# Autodesk Inventor assembly: pinballAssembly
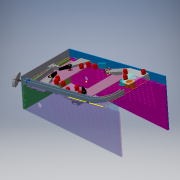
[picture p0: Inventor's stored thumbnail of the model, 180x180]
Saved by Autodesk Inventor 2017 (Build 210142000, 142)
## iProperties
Created: 2017-02-19
Part Number: pinballAssembly
Document SubType Name: Assembly
Designer: John
Author: John
## Documents named in this file (34)
- C:\Users\John\Dropbox\ECE115\pinball-project\pinballAssembly.iam
- C:\Users\John\Dropbox\ECE115\pinball-project\playfield.ipt
- C:\Users\John\Dropbox\ECE115\pinball-project\modular-post.ipt
- C:\Users\John\Dropbox\ECE115\module-2\paddle2.ipt
- C:\Users\John\Dropbox\ECE115\pinball-project\part_pinball_ece115.ipt
- C:\Users\John\Dropbox\ECE115\pinball-project\flipper-hug-left.ipt
- C:\Users\John\Dropbox\ECE115\pinball-project\thumper-bumper-assm-v3.iam
- C:\Users\John\Dropbox\ECE115\pinball-project\pinball-case-left-wall.ipt
- C:\Users\John\Dropbox\ECE115\pinball-project\pinball-case-left-wall-outer.ipt
- C:\Users\John\Dropbox\ECE115\pinball-project\wall-front.ipt
- C:\Users\John\Dropbox\ECE115\pinball-project\wall-front-outer.ipt
- C:\Users\John\Dropbox\ECE115\pinball-project\plunger-curve-outer.ipt
- C:\Users\John\Dropbox\ECE115\pinball-project\plunger-curve-inner.ipt
- C:\Users\John\Dropbox\ECE115\pinball-project\ball-reload-right.ipt
- C:\Users\John\Dropbox\ECE115\pinball-project\ball-waterfall.ipt
- C:\Users\John\Dropbox\ECE115\pinball-project\ramp-support.ipt
- C:\Users\John\Dropbox\ECE115\pinball-project\flipper-support.ipt
- C:\Users\John\Dropbox\ECE115\module-2\rod.ipt
- C:\Users\John\Dropbox\ECE115\module-2\Solenoid 1240S\Solenoid.iam
- C:\Users\John\Dropbox\ECE115\pinball-project\pinball-case-back.ipt
- C:\Users\John\Dropbox\ECE115\pinball-project\game-over.ipt
- C:\Users\John\Dropbox\ECE115\pinball-project\flipper-hug-left-2.ipt
- C:\Users\John\Downloads\level2.ipt
- C:\Users\John\Downloads\funil.ipt
- C:\Users\John\Downloads\ramp.ipt
- C:\Users\John\Downloads\ServoMotor.ipt
- C:\Users\John\Downloads\GATE servo motor.ipt
- C:\Users\John\Downloads\wall-outer-plunger-updated.ipt
- C:\Users\John\Downloads\wall-inner-plunger-updated.ipt
- C:\Users\John\Downloads\plunger-support.ipt
- C:\Users\John\Downloads\Handle_plunger.ipt
- C:\Users\John\Dropbox\ECE115\pinball-project\flipper-support2.ipt
- C:\Users\John\Dropbox\ECE115\module-2\flipper-bottom.ipt
- C:\Users\John\Dropbox\ECE115\module-2\interstitial-flipper.ipt
## Components (59 placed, 33 different names)
1. playfield:1 — Mate:1, Mate:2, Tangent:1, Mate:10, Insert:4, Insert:5, Insert:6, Flush:8, Mate:16, Flush:18, Tangent:3, Mate:29, Mate:30, Mate:31, Mate:34, Mate:41, Angle:8, Mate:42, Mate:50, Mate:51, Mate:54, Mate:55, Angle:12, Angle:13, Angle:14, Mate:65, Mate:66, Flush:34, Mate:67, Mate:68, Mate:69, Mate:76, Angle:17, Flush:35, Mate:80, Angle:18, Mate:83, Mate:85, Mate:86, Mate:87, Flush:36, Mate:88, Mate:89, Mate:90, Mate:96, Rotational:11, Mate:121, Mate:122, Mate:123
2. modular-post:1 — Insert:5
3. modular-post:2 — Insert:4
4. modular-post:3 — Insert:6
5. paddle2:1 — Mate:1, Mate:55, Mate:56, Mate:77
6. paddle2:2 — Mate:2, Rotational:4, Mate:54, Mate:57, Flush:31
7. part_pinball_ece115:1 — Tangent:1
8. flipper-hug-left:2 — Mate:10, Rotational:4, Angle:12
9. modular-post:4
10. modular-post:5
11. modular-post:6
12. thumper-bumper-assm-v3:1 [sub-assembly] — Mate:65, Mate:66, Flush:34
13. thumper-bumper-assm-v3:2 [sub-assembly] — Flush:8, Mate:67, Mate:68
14. pinball-case-left-wall:1 — Mate:16, Flush:23, Flush:24, Flush:25, Mate:47, Flush:29, Mate:49, Mate:50, Mate:51, Flush:30, Mate:52, Mate:53, Angle:19, Mate:102, Mate:104, Mate:105
15. pinball-case-left-wall-outer:1 — Flush:25, Mate:47, Flush:26, Flush:27, Angle:15, Mate:79, Mate:82
16. wall-front:1 — Flush:15, Flush:17, Mate:22, Flush:23, Flush:24, Flush:28, Mate:48, Mate:49, Angle:21
17. pinball-case-left-wall-outer:2 — Flush:15, Tangent:2, Angle:4, Tangent:4, Flush:27, Mate:75
18. wall-front-outer:1 — Flush:17, Flush:18, Mate:22, Flush:26
19. plunger-curve-outer:1 — Tangent:2, Angle:4, Tangent:3, Angle:5, Flush:22
20. plunger-curve-inner:1 — Angle:5, Tangent:4, Flush:22
21. modular-post:7 — Mate:29
22. modular-post:8 — Mate:30
23. modular-post:10 — Mate:31
24. paddle2:3 — Mate:34, Mate:101, Flush:38, Rotational:11
25. ball-reload-right:1 — Mate:121, Mate:122, Mate:123
26. ball-waterfall:1 — Mate:41, Angle:8, Mate:78
27. ramp-support:1 — Mate:42, Flush:39, Mate:106
28. pinball-case-left-wall:2 — Flush:28, Flush:29, Mate:48, Flush:32, Mate:61, Mate:62, Mate:75
29. flipper-support:1 — Flush:30, Mate:52, Mate:53, Mate:59, Mate:109, Mate:110
30. rod:1 — Mate:57, Flush:31, Mate:112
31. rod:2 — Mate:56, Mate:115
32. Solenoid:1 [sub-assembly] — Mate:59, Angle:13, Mate:109, Rotational:13
33. pinball-case-back:1 — Angle:14, Flush:32, Mate:61, Mate:62
34. game-over:1 — Mate:69, Angle:15
35. flipper-hug-left-2:1 — Mate:76, Angle:17, Mate:77
36. level2:1 — Mate:78, Mate:79, Flush:35, Mate:81, Rotational:7, Rotational:8, Rotational:9, Mate:84
37. funil:1 — Mate:80, Mate:81, Angle:18
38. modular-post:12 — Rotational:7
39. modular-post:13 — Rotational:8
40. modular-post:14 — Rotational:9
41. ramp:1 — Mate:82, Mate:83, Mate:84, Flush:39, Mate:106
42. ServoMotor:1 — Mate:85, Angle:19, Mate:86, Rotational:10
43. GATE servo motor:1 — Rotational:10
44. wall-outer-plunger-updated:1 — Mate:87, Flush:36, Mate:88, Mate:91, Mate:93, Mate:94, Flush:37
45. wall-inner-plunger-updated:1 — Mate:89, Mate:90, Mate:91
46. plunger-support:1 — Mate:93, Mate:94, Flush:37, Mate:95, Angle:20
47. Handle_plunger:1 — Mate:95, Angle:20, Mate:96, Mate:97, Mate:98
48. rod:3 — Mate:97, Mate:98, Mate:99, Mate:100
49. rod:4 — Mate:99, Mate:100
50. rod:5 — Mate:101, Flush:38, Mate:118
51. flipper-support2:1 — Mate:102, Mate:104, Mate:105, Mate:111
52. Solenoid:2 [sub-assembly] — Mate:110, Angle:21, Rotational:12
53. Solenoid:3 [sub-assembly] — Mate:111, Rotational:14
54. flipper-bottom:1 — Mate:115, Mate:116, Mate:117
55. flipper-bottom:2 — Mate:112, Mate:113, Mate:114
56. flipper-bottom:3 — Mate:118, Mate:119, Mate:120
57. interstitial-flipper:1 — Rotational:12, Mate:113, Mate:114
58. interstitial-flipper:2 — Rotational:14, Mate:119, Mate:120
59. interstitial-flipper:3 — Rotational:13, Mate:116, Mate:117
## Relationships (124: Mate 75, Flush 21, Angle 12, RevoluteJoint 9, Tangent 4, Insert 3)
- Mate:1: playfield:1 ↔ paddle2:1
- Mate:2: playfield:1 ↔ paddle2:2
- Tangent:1: playfield:1 ↔ part_pinball_ece115:1
- Mate:10: playfield:1 ↔ flipper-hug-left:2
- Rotational:4 [RevoluteJoint]: paddle2:2 ↔ flipper-hug-left:2
- Insert:4: playfield:1 ↔ modular-post:2
- Insert:5: playfield:1 ↔ modular-post:1
- Insert:6: playfield:1 ↔ modular-post:3
- Flush:8: playfield:1 ↔ thumper-bumper-assm-v3:2
- Mate:16: playfield:1 ↔ pinball-case-left-wall:1
- Flush:15: wall-front:1 ↔ pinball-case-left-wall-outer:2
- Flush:17: wall-front:1 ↔ wall-front-outer:1
- Flush:18 (-3 mm): playfield:1 ↔ wall-front-outer:1
- Mate:22: wall-front:1 ↔ wall-front-outer:1
- Tangent:2: pinball-case-left-wall-outer:2 ↔ plunger-curve-outer:1
- Angle:4 (90 deg): pinball-case-left-wall-outer:2 ↔ plunger-curve-outer:1
- Tangent:3: playfield:1 ↔ plunger-curve-outer:1
- Angle:5 (0 deg): plunger-curve-outer:1 ↔ plunger-curve-inner:1
- Tangent:4 (20 mm): pinball-case-left-wall-outer:2 ↔ plunger-curve-inner:1
- Flush:22: plunger-curve-outer:1 ↔ plunger-curve-inner:1
- Mate:29: playfield:1 ↔ modular-post:7
- Mate:30: playfield:1 ↔ modular-post:8
- Mate:31: playfield:1 ↔ modular-post:10
- Mate:34: playfield:1 ↔ paddle2:3
- Mate:41: playfield:1 ↔ ball-waterfall:1
- Angle:8 (15 deg): playfield:1 ↔ ball-waterfall:1
- Mate:42: playfield:1 ↔ ramp-support:1
- Flush:23: pinball-case-left-wall:1 ↔ wall-front:1
- Flush:24: pinball-case-left-wall:1 ↔ wall-front:1
- Flush:25: pinball-case-left-wall:1 ↔ pinball-case-left-wall-outer:1
- Mate:47: pinball-case-left-wall:1 ↔ pinball-case-left-wall-outer:1
- Flush:26 (3 mm): pinball-case-left-wall-outer:1 ↔ wall-front-outer:1
- Flush:27: pinball-case-left-wall-outer:1 ↔ pinball-case-left-wall-outer:2
- Flush:28: wall-front:1 ↔ pinball-case-left-wall:2
- Flush:29: pinball-case-left-wall:1 ↔ pinball-case-left-wall:2
- Mate:48: wall-front:1 ↔ pinball-case-left-wall:2
- Mate:49: pinball-case-left-wall:1 ↔ wall-front:1
- Mate:50: playfield:1 ↔ pinball-case-left-wall:1
- Mate:51: playfield:1 ↔ pinball-case-left-wall:1
- Flush:30: pinball-case-left-wall:1 ↔ flipper-support:1
- Mate:52: pinball-case-left-wall:1 ↔ flipper-support:1
- Mate:53: pinball-case-left-wall:1 ↔ flipper-support:1
- Mate:54: playfield:1 ↔ paddle2:2
- Mate:55: playfield:1 ↔ paddle2:1
- Angle:12 (0 deg): playfield:1 ↔ flipper-hug-left:2
- Mate:56: paddle2:1 ↔ rod:2
- Mate:57: paddle2:2 ↔ rod:1
- Flush:31: paddle2:2 ↔ rod:1
- Mate:59: flipper-support:1 ↔ Solenoid:1
- Angle:13 (180 deg): playfield:1 ↔ Solenoid:1
- Angle:14 (0 deg): playfield:1 ↔ pinball-case-back:1
- Flush:32: pinball-case-left-wall:2 ↔ pinball-case-back:1
- Mate:61: pinball-case-left-wall:2 ↔ pinball-case-back:1
- Mate:62: pinball-case-left-wall:2 ↔ pinball-case-back:1
- Mate:65: playfield:1 ↔ thumper-bumper-assm-v3:1
- Mate:66: playfield:1 ↔ thumper-bumper-assm-v3:1
- Flush:34: playfield:1 ↔ thumper-bumper-assm-v3:1
- Mate:67: playfield:1 ↔ thumper-bumper-assm-v3:2
- Mate:68: playfield:1 ↔ thumper-bumper-assm-v3:2
- Mate:69: playfield:1 ↔ game-over:1
- Angle:15 (180 deg): pinball-case-left-wall-outer:1 ↔ game-over:1
- Mate:75: pinball-case-left-wall-outer:2 ↔ pinball-case-left-wall:2
- Mate:76: playfield:1 ↔ flipper-hug-left-2:1
- Angle:17 (0 deg): playfield:1 ↔ flipper-hug-left-2:1
- Mate:77: paddle2:1 ↔ flipper-hug-left-2:1
- Mate:78 (3 mm): ball-waterfall:1 ↔ level2:1
- Mate:79: pinball-case-left-wall-outer:1 ↔ level2:1
- Flush:35: playfield:1 ↔ level2:1
- Mate:80: playfield:1 ↔ funil:1
- Mate:81: level2:1 ↔ funil:1
- Angle:18 (100 deg): playfield:1 ↔ funil:1
- Rotational:7 [RevoluteJoint]: level2:1 ↔ modular-post:12
- Rotational:8 [RevoluteJoint]: level2:1 ↔ modular-post:13
- Rotational:9 [RevoluteJoint]: level2:1 ↔ modular-post:14
- Mate:82: pinball-case-left-wall-outer:1 ↔ ramp:1
- Mate:83: playfield:1 ↔ ramp:1
- Mate:84: level2:1 ↔ ramp:1
- Mate:85: playfield:1 ↔ ServoMotor:1
- Angle:19 (0 deg): pinball-case-left-wall:1 ↔ ServoMotor:1
- Mate:86: playfield:1 ↔ ServoMotor:1
- Rotational:10 [RevoluteJoint]: ServoMotor:1 ↔ GATE servo motor:1
- Mate:87: playfield:1 ↔ wall-outer-plunger-updated:1
- Flush:36: playfield:1 ↔ wall-outer-plunger-updated:1
- Mate:88: playfield:1 ↔ wall-outer-plunger-updated:1
- Mate:89: playfield:1 ↔ wall-inner-plunger-updated:1
- Mate:90: playfield:1 ↔ wall-inner-plunger-updated:1
- Mate:91 (14 mm): wall-outer-plunger-updated:1 ↔ wall-inner-plunger-updated:1
- Mate:93: wall-outer-plunger-updated:1 ↔ plunger-support:1
- Mate:94: wall-outer-plunger-updated:1 ↔ plunger-support:1
- Flush:37: wall-outer-plunger-updated:1 ↔ plunger-support:1
- Mate:95: plunger-support:1 ↔ Handle_plunger:1
- Angle:20 (180 deg): plunger-support:1 ↔ Handle_plunger:1
- Mate:96 (40 mm): playfield:1 ↔ Handle_plunger:1
- Mate:97: Handle_plunger:1 ↔ rod:3
- Mate:98: Handle_plunger:1 ↔ rod:3
- Mate:99: rod:3 ↔ rod:4
- Mate:100: rod:3 ↔ rod:4
- Mate:101: paddle2:3 ↔ rod:5
- Flush:38: paddle2:3 ↔ rod:5
- Rotational:11 [RevoluteJoint]: playfield:1 ↔ paddle2:3
- Mate:102: pinball-case-left-wall:1 ↔ flipper-support2:1
- Mate:104: pinball-case-left-wall:1 ↔ flipper-support2:1
- Mate:105: pinball-case-left-wall:1 ↔ flipper-support2:1
- Flush:39: ramp-support:1 ↔ ramp:1
- Mate:106: ramp-support:1 ↔ ramp:1
- Mate:109: flipper-support:1 ↔ Solenoid:1
- Mate:110: flipper-support:1 ↔ Solenoid:2
- Angle:21 (180 deg): wall-front:1 ↔ Solenoid:2
- Mate:111: flipper-support2:1 ↔ Solenoid:3
- Mate:112: rod:1 ↔ flipper-bottom:2
- Rotational:12 [RevoluteJoint]: Solenoid:2 ↔ interstitial-flipper:1
- Mate:113: flipper-bottom:2 ↔ interstitial-flipper:1
- Mate:114: flipper-bottom:2 ↔ interstitial-flipper:1
- Rotational:13 [RevoluteJoint]: Solenoid:1 ↔ interstitial-flipper:3
- Mate:115: rod:2 ↔ flipper-bottom:1
- Mate:116: flipper-bottom:1 ↔ interstitial-flipper:3
- Mate:117: flipper-bottom:1 ↔ interstitial-flipper:3
- Rotational:14 [RevoluteJoint]: Solenoid:3 ↔ interstitial-flipper:2
- Mate:118: rod:5 ↔ flipper-bottom:3
- Mate:119: flipper-bottom:3 ↔ interstitial-flipper:2
- Mate:120: flipper-bottom:3 ↔ interstitial-flipper:2
- Mate:121: playfield:1 ↔ ball-reload-right:1
- Mate:122: playfield:1 ↔ ball-reload-right:1
- Mate:123: playfield:1 ↔ ball-reload-right:1
